# Autodesk Inventor assembly: Durometer_Electronics_Enclosure_Assembly
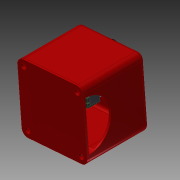
[picture p0: Inventor's stored thumbnail of the model, 180x180]
Saved by Autodesk Inventor 2015 (Build 190159000, 159)
## iProperties
Created: 2015-01-04
Part Number: Durometer_Electronics_Enclosure_Assembly
Document SubType Name: Assembly
Designer: Drew
Author: Drew
## Documents named in this file (6)
- C:\Users\Drew\Dropbox\Durometer\Durometer_Assembly\Durometer_Electronics_Enclosure_Assembly.iam
- C:\Users\Drew\Dropbox\Durometer\Durometer_Assembly\Durometer_Electronics_Enclosure.ipt
- C:\Users\Drew\Dropbox\Durometer\Durometer_Assembly\Arduino_pro_mini.iam
- C:\Users\Drew\Dropbox\Durometer\Durometer_Assembly\Big_Easy_Stepper_Driver.ipt
- C:\Users\Drew\Dropbox\Durometer\Durometer_Assembly\MB2011SS1W01_CA.iam
- C:\Users\Drew\Dropbox\Durometer\Durometer_Assembly\Durometer_Electronics_Enclosure_Lid.ipt
## Components (6 placed, 5 different names)
1. Durometer_Electronics_Enclosure:1 — Mate:1, Mate:2, Mate:9, Mate:10, Mate:11, Mate:12, Mate:13, Mate:14
2. Arduino_pro_mini:1 [sub-assembly] — Mate:2, Mate:14
3. Big_Easy_Stepper_Driver:1 — Mate:1, Mate:12, Mate:13
4. MB2011SS1W01_CA:1 [sub-assembly] — Mate:5, Mate:7
5. MB2011SS1W01_CA:2 [sub-assembly] — Mate:6, Mate:8
6. Durometer_Electronics_Enclosure_Lid:1 — Mate:5, Mate:6, Mate:7, Mate:8, Mate:9, Mate:10, Mate:11
## Relationships (12: Mate 12)
- Mate:1: Durometer_Electronics_Enclosure:1 ↔ Big_Easy_Stepper_Driver:1
- Mate:2: Durometer_Electronics_Enclosure:1 ↔ Arduino_pro_mini:1
- Mate:5: MB2011SS1W01_CA:1 ↔ Durometer_Electronics_Enclosure_Lid:1
- Mate:6: MB2011SS1W01_CA:2 ↔ Durometer_Electronics_Enclosure_Lid:1
- Mate:7: MB2011SS1W01_CA:1 ↔ Durometer_Electronics_Enclosure_Lid:1
- Mate:8: MB2011SS1W01_CA:2 ↔ Durometer_Electronics_Enclosure_Lid:1
- Mate:9: Durometer_Electronics_Enclosure:1 ↔ Durometer_Electronics_Enclosure_Lid:1
- Mate:10: Durometer_Electronics_Enclosure:1 ↔ Durometer_Electronics_Enclosure_Lid:1
- Mate:11: Durometer_Electronics_Enclosure:1 ↔ Durometer_Electronics_Enclosure_Lid:1
- Mate:12: Durometer_Electronics_Enclosure:1 ↔ Big_Easy_Stepper_Driver:1
- Mate:13: Durometer_Electronics_Enclosure:1 ↔ Big_Easy_Stepper_Driver:1
- Mate:14 (-38.1 mm): Durometer_Electronics_Enclosure:1 ↔ Arduino_pro_mini:1
